# Autodesk Inventor assembly: CAD_1
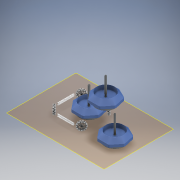
[picture p0: Inventor's stored thumbnail of the model, 180x180]
Saved by Autodesk Inventor 2022 (Build 260153000, 153)
## iProperties
Created: 2021-05-23
Part Number: CAD_1
Document SubType Name: Assembly
Designer: carlo
Author: carlo
## Documents named in this file (5)
- C:\the7dorks.github.io\CAD_1.iam
- C:\the7dorks.github.io\Library 1.2\Motion\Wheels\Omnis\4 Omni, Square.ipt
- C:\the7dorks.github.io\Library 1.2\Structure\C-Channels\Aluminum 1x2x1\1x2x1x16 Aluminum.ipt
- C:\the7dorks.github.io\Tipping Poing Field CAD\Alliance_Mobile_Goal_Blue.iam
- C:\the7dorks.github.io\Tipping Poing Field CAD\Neutral_Mobile_Goal_Short.iam
## Components (14 placed, 4 different names)
1. 4 Omni, Square:1
2. 4 Omni, Square:2
3. 4 Omni, Square:3
4. 4 Omni, Square:4
5. 1x2x1x16 Aluminum:1
6. Alliance_Mobile_Goal_Blue:1 [sub-assembly]
7. Alliance_Mobile_Goal_Blue:2 [sub-assembly]
8. Alliance_Mobile_Goal_Blue:3 [sub-assembly]
9. 1x2x1x16 Aluminum:2
10. 1x2x1x16 Aluminum:3
11. Neutral_Mobile_Goal_Short:1 [sub-assembly]
12. Alliance_Mobile_Goal_Blue:4 [sub-assembly]
13. Alliance_Mobile_Goal_Blue:5 [sub-assembly]
14. Alliance_Mobile_Goal_Blue:6 [sub-assembly]
## Relationships (6: Flush 6)
- Flush:1 (228.6 mm)
- Flush:2 (-228.6 mm)
- Flush:3 (228.6 mm)
- Flush:4 (-228.6 mm)
- Flush:5 (457.2 mm)
- Flush:6
